# Autodesk Inventor assembly: EngineAssembly
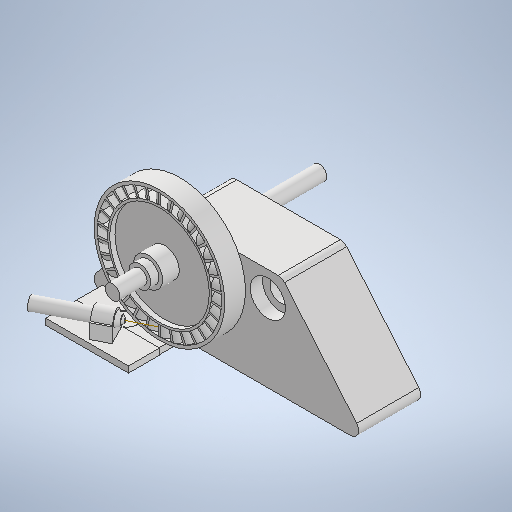
[picture p0: Inventor's stored thumbnail of the model, 512x512]
Saved by Autodesk Inventor 2026.1 (Build 301233020, 233B)
## iProperties
Created: 2025-10-27
Part Number: EngineAssembly
Document SubType Name: Assembly
Designer: yo
Author: yo
## Documents named in this file (6)
- C:\Users\yo\Documents\Andes\9no Semestre\Proyecto Intermedio\Proyecto\Huron-Hudson\Pelton Engine\V8\EngineAssembly.iam
- C:\Users\yo\Documents\Andes\9no Semestre\Proyecto Intermedio\Proyecto\Huron-Hudson\Pelton Engine\V8\EngineMount.ipt
- C:\Users\yo\Documents\Andes\9no Semestre\Proyecto Intermedio\Proyecto\Huron-Hudson\Pelton Engine\V8\Shaft.ipt
- C:\Users\yo\Documents\Andes\9no Semestre\Proyecto Intermedio\Proyecto\Huron-Hudson\Pelton Engine\V8\Turbine-V5.ipt
- C:\Users\yo\Documents\Andes\9no Semestre\Proyecto Intermedio\Proyecto\Huron-Hudson\Pelton Engine\V8\Nozzle Fixer.ipt
- C:\Users\yo\Documents\Andes\9no Semestre\Proyecto Intermedio\Proyecto\Huron-Hudson\Pelton Engine\V8\Nozzle.ipt
## Components (5 placed, 5 different names)
1. EngineMount:1 — Flush:1, Flush:2, Flush:3, Mate:1, Mate:2, Tangent:1, Flush:4, Tangent:2, Mate:4
2. Shaft:1 — Mate:1, Mate:2, Mate:3
3. Turbine-V5:1 — Mate:3, Tangent:1
4. Nozzle Fixer:1 — Flush:4, Tangent:2, Mate:4, Mate:5, Mate:6, Tangent:3
5. Nozzle:1 — Mate:6, Tangent:3
## Relationships (13: Mate 6, Flush 4, Tangent 3)
- Flush:1: EngineMount:1
- Flush:2: EngineMount:1
- Flush:3: EngineMount:1
- Mate:1: EngineMount:1 ↔ Shaft:1
- Mate:2: EngineMount:1 ↔ Shaft:1
- Mate:3: Shaft:1 ↔ Turbine-V5:1
- Tangent:1: EngineMount:1 ↔ Turbine-V5:1
- Flush:4: EngineMount:1 ↔ Nozzle Fixer:1
- Tangent:2: EngineMount:1 ↔ Nozzle Fixer:1
- Mate:4: EngineMount:1 ↔ Nozzle Fixer:1
- Mate:5: Nozzle Fixer:1
- Mate:6: Nozzle Fixer:1 ↔ Nozzle:1
- Tangent:3: Nozzle Fixer:1 ↔ Nozzle:1
